# Autodesk Inventor assembly: Ensamblaje1
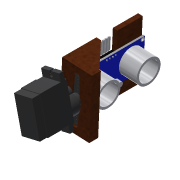
[picture p0: Inventor's stored thumbnail of the model, 180x180]
Saved by Autodesk Inventor 2016 (Build 200138000, 138)
## iProperties
Created: 2016-08-02
Part Number: Ensamblaje1
Material: Genérico
Document SubType Name: Assembly
Designer: DanielFelipe
Author: DanielFelipe
## Documents named in this file (7)
- C:\Users\julianesteban\Documents\MEGA\Julián y Espitia\diseños inventor elementos comerciales\ultrasonico HC-SR04\ensamble total\Ensamblaje1.iam
- C:\Users\julianesteban\Documents\MEGA\Julián y Espitia\diseños inventor elementos comerciales\ultrasonico HC-SR04\ensamble total\PARTE 1.ipt
- C:\Users\julianesteban\Documents\MEGA\Julián y Espitia\diseños inventor elementos comerciales\ultrasonico HC-SR04\ensamble total\acople madera.ipt
- C:\Users\julianesteban\Documents\MEGA\Julián y Espitia\diseños inventor elementos comerciales\ultrasonico HC-SR04\ensamble total\acople 2.ipt
- C:\Users\julianesteban\Documents\MEGA\Julián y Espitia\diseños inventor elementos comerciales\ultrasonico HC-SR04\ensamble total\acople 3.ipt
- C:\Users\julianesteban\Documents\MEGA\Julián y Espitia\diseños inventor elementos comerciales\ultrasonico HC-SR04\ensamble total\acople 4.ipt
- C:\Users\julianesteban\Documents\MEGA\Julián y Espitia\diseños inventor elementos comerciales\ultrasonico HC-SR04\ensamble total\servo motor MG90S\ensamble.iam
## Components (7 placed, 6 different names)
1. PARTE 1:1 — Nivelación:2, Coincidencia:5, Mate:14
2. acople madera:1 — Nivelación:2, Coincidencia:4, Nivelación:3, Nivelación:4, Coincidencia:6, Mate:11, Mate:12
3. acople 2:1 — Coincidencia:4, Nivelación:3, Nivelación:4, Coincidencia:5, Nivelación:5, Nivelación:6, Coincidencia:7, Nivelación:7, Coincidencia:9, Nivelación:8, Mate:13
4. acople 3:1 — Coincidencia:6, Nivelación:5, Nivelación:6, Coincidencia:8, Coincidencia:10, Mate:14
5. acople 4:1 — Coincidencia:7, Coincidencia:8, Nivelación:7
6. acople 4:2 — Coincidencia:9, Coincidencia:10, Nivelación:8
7. ensamble:1 [sub-assembly] — Mate:11, Mate:12, Mate:13
## Relationships (18: Mate 11, Flush 7)
- Nivelación:2 [Flush] (15 mm): PARTE 1:1 ↔ acople madera:1
- Coincidencia:4 [Mate]: acople madera:1 ↔ acople 2:1
- Nivelación:3 [Flush]: acople madera:1 ↔ acople 2:1
- Nivelación:4 [Flush]: acople madera:1 ↔ acople 2:1
- Coincidencia:5 [Mate]: PARTE 1:1 ↔ acople 2:1
- Coincidencia:6 [Mate]: acople madera:1 ↔ acople 3:1
- Nivelación:5 [Flush]: acople 2:1 ↔ acople 3:1
- Nivelación:6 [Flush]: acople 2:1 ↔ acople 3:1
- Coincidencia:7 [Mate]: acople 2:1 ↔ acople 4:1
- Coincidencia:8 [Mate]: acople 3:1 ↔ acople 4:1
- Nivelación:7 [Flush]: acople 2:1 ↔ acople 4:1
- Coincidencia:9 [Mate]: acople 2:1 ↔ acople 4:2
- Coincidencia:10 [Mate]: acople 3:1 ↔ acople 4:2
- Nivelación:8 [Flush]: acople 2:1 ↔ acople 4:2
- Mate:11: acople madera:1 ↔ ensamble:1
- Mate:12: acople madera:1 ↔ ensamble:1
- Mate:13: acople 2:1 ↔ ensamble:1
- Mate:14 (2.04 mm): PARTE 1:1 ↔ acople 3:1
